# Autodesk Inventor assembly: actuator
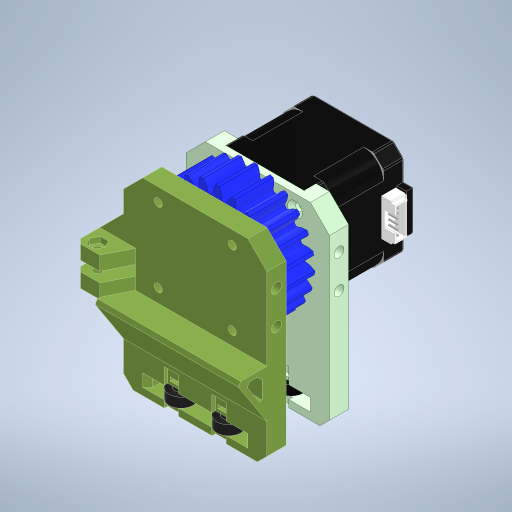
[picture p0: Inventor's stored thumbnail of the model, 512x512]
Saved by Autodesk Inventor 2023.1 (Build 271208000, 208)
## iProperties
Created: 2025-12-13
Part Number: actuator
Document SubType Name: Assembly
Designer: DELL
Author: DELL
## Documents named in this file (8)
- C:\Users\DELL\reposGitHub\VSOSH25-26\models\actuator\actuator_actual\actuator.iam
- C:\Users\DELL\reposGitHub\VSOSH25-26\models\actuator\actuator_actual\Schrittmotor-42SHDC3025-24B.ipt
- C:\Users\DELL\reposGitHub\VSOSH25-26\models\actuator\actuator_actual\звезда_шестрерни.ipt
- C:\Users\DELL\reposGitHub\VSOSH25-26\models\actuator\actuator_actual\муфта.ipt
- C:\Users\DELL\reposGitHub\VSOSH25-26\models\actuator\actuator_actual\шестреня_12.12.ipt
- C:\Users\DELL\reposGitHub\VSOSH25-26\models\actuator\actuator_actual\каретка.ipt
- C:\Users\DELL\reposGitHub\VSOSH25-26\models\actuator\actuator_actual\колесико.ipt
- C:\Users\DELL\reposGitHub\VSOSH25-26\models\actuator\actuator_actual\каретка_м3_без_м.ipt
## Components (10 placed, 7 different names)
1. Schrittmotor-42SHDC3025-24B:1 — Заподлицо:1, Совмещение:1, Совмещение:2, Совмещение:4, Заподлицо:3, Совмещение:62, Совмещение:63
2. звезда_шестрерни:1 — Совмещение:5, Совмещение:6, Совмещение:7, Совмещение:8, Заподлицо:2
3. муфта:1 — Совмещение:4, Совмещение:5, Совмещение:6, Совмещение:9
4. шестреня_12.12:1 — Совмещение:7, Совмещение:8, Заподлицо:2
5. каретка:1 — Заподлицо:3, Совмещение:9, Совмещение:41, Совмещение:53, Заподлицо:5, Заподлицо:6, Совмещение:62, Совмещение:63
6. колесико:2 — Совмещение:53
7. колесико:6 — Совмещение:41
8. каретка_м3_без_м:1 — Совмещение:57, Совмещение:58, Совмещение:59, Совмещение:60, Заподлицо:5, Заподлицо:6
9. колесико:7 — Совмещение:59, Совмещение:60
10. колесико:8 — Совмещение:57, Совмещение:58
## Relationships (21: Mate 16, Flush 5)
- Заподлицо:1 [Flush]: Schrittmotor-42SHDC3025-24B:1
- Совмещение:1 [Mate]: Schrittmotor-42SHDC3025-24B:1
- Совмещение:2 [Mate]: Schrittmotor-42SHDC3025-24B:1
- Совмещение:4 [Mate]: Schrittmotor-42SHDC3025-24B:1 ↔ муфта:1
- Совмещение:5 [Mate]: звезда_шестрерни:1 ↔ муфта:1
- Совмещение:6 [Mate]: звезда_шестрерни:1 ↔ муфта:1
- Совмещение:7 [Mate]: звезда_шестрерни:1 ↔ шестреня_12.12:1
- Совмещение:8 [Mate]: звезда_шестрерни:1 ↔ шестреня_12.12:1
- Заподлицо:2 [Flush]: звезда_шестрерни:1 ↔ шестреня_12.12:1
- Заподлицо:3 [Flush]: Schrittmotor-42SHDC3025-24B:1 ↔ каретка:1
- Совмещение:9 [Mate]: муфта:1 ↔ каретка:1
- Совмещение:41 [Mate]: каретка:1 ↔ колесико:6
- Совмещение:53 [Mate]: каретка:1 ↔ колесико:2
- Совмещение:57 [Mate]: каретка_м3_без_м:1 ↔ колесико:8
- Совмещение:58 [Mate]: каретка_м3_без_м:1 ↔ колесико:8
- Совмещение:59 [Mate]: каретка_м3_без_м:1 ↔ колесико:7
- Совмещение:60 [Mate]: каретка_м3_без_м:1 ↔ колесико:7
- Заподлицо:5 [Flush]: каретка:1 ↔ каретка_м3_без_м:1
- Заподлицо:6 [Flush]: каретка:1 ↔ каретка_м3_без_м:1
- Совмещение:62 [Mate]: Schrittmotor-42SHDC3025-24B:1 ↔ каретка:1
- Совмещение:63 [Mate]: Schrittmotor-42SHDC3025-24B:1 ↔ каретка:1
